# Autodesk Inventor assembly: KnopfZusammenbau
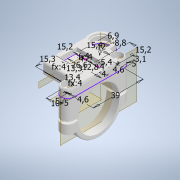
[picture p0: Inventor's stored thumbnail of the model, 180x180]
Saved by Autodesk Inventor 2020.2 (Build 242310000, 310)
## iProperties
Created: 2020-05-20
Part Number: KnopfZusammenbau
Document SubType Name: Assembly
Designer: hpcwoess
Author: hpcwoess
## Documents named in this file (4)
- C:\Users\Uwe\3DDrucke\OpenBikeSensor\KnopfZusammenbau.iam
- C:\Users\Uwe\3DDrucke\OpenBikeSensor\Oberschale.ipt
- C:\Users\Uwe\3DDrucke\OpenBikeSensor\Zwischenstueck.ipt
- C:\Users\Uwe\3DDrucke\OpenBikeSensor\Schelle32.ipt
## Components (3 placed, 3 different names)
1. Oberschale:1 — Fluchtend:1, Fluchtend:3, Passend:1
2. Zwischenstueck:1 — Fluchtend:5, Fluchtend:6, Fluchtend:7, Passend:1, Passend:2, Passend:3
3. Schelle32:1 — Passend:2, Passend:3
## Relationships (8: Flush 5, Mate 3)
- Fluchtend:1 [Flush]: Oberschale:1
- Fluchtend:3 [Flush]: Oberschale:1
- Fluchtend:5 [Flush]: Zwischenstueck:1
- Fluchtend:6 [Flush]: Zwischenstueck:1
- Fluchtend:7 [Flush]: Zwischenstueck:1
- Passend:1 [Mate]: Oberschale:1 ↔ Zwischenstueck:1
- Passend:2 [Mate] (2 mm): Zwischenstueck:1 ↔ Schelle32:1
- Passend:3 [Mate]: Zwischenstueck:1 ↔ Schelle32:1
